# Autodesk Inventor assembly: BNT 2010-2.6 +1166L C7T-J1K_10000KBK 15BF 15
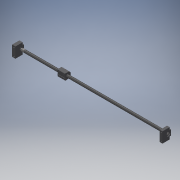
[picture p0: Inventor's stored thumbnail of the model, 180x180]
Saved by Autodesk Inventor 2018 (Build 220112000, 112)
## iProperties
Category: PARTsolutions
Company: THK
Created: 2017-05-30
Part Number: BNT 2010-2.6 +1166L C7T-J1K_10000KBK 15BF 15
Catalog Web Link: www.cadenas.de
Description: Rectangular-Nut Non-Preloaded Type BNT-
Vendor: THK
Document SubType Name: Assembly
Designer: psAdmin
Manufacturer: THK
Title: BNT 2010-2.6 +1166L C7T-J1K
Author: Cadenas PARTsolutions
## Documents named in this file (7)
- C:\Users\P300023\Documents\GitHub\CNC-Lathe-CAD2.0\CNC Lathe Project\Project Files\Updated Z axis\AIS2016\Z-AxisLong-Shaft-Final.iam
- C:\Users\P300023\Documents\GitHub\CNC-Lathe-CAD2.0\CNC Lathe Project\Project Files\Updated Z axis\AIS2016\BNT 2010-2_61000-J1K Shaft.ipt
- C:\Users\P300023\Documents\GitHub\CNC-Lathe-CAD2.0\CNC Lathe Project\Project Files\Updated Z axis\AIS2016\BNT 2010-2_6 Nut.ipt
- C:\Users\P300023\Documents\GitHub\CNC-Lathe-CAD2.0\CNC Lathe Project\Project Files\Updated Z axis\AIS2016\BK 15.ipt
- C:\Users\P300023\Documents\GitHub\CNC-Lathe-CAD2.0\CNC Lathe Project\Project Files\Updated Z axis\AIS2016\BK 15collar.ipt
- C:\Users\P300023\Documents\GitHub\CNC-Lathe-CAD2.0\CNC Lathe Project\Project Files\Updated Z axis\AIS2016\BF 15 Part2.ipt
- C:\Users\P300023\Documents\GitHub\CNC-Lathe-CAD2.0\CNC Lathe Project\Project Files\Updated Z axis\AIS2016\BF 15 Part1.ipt
## Components (6 placed, 6 different names)
1. BNT 2010-2_61000-J1K Shaft:1 — Mate:1
2. BNT 2010-2_6 Nut:1 — Mate:1
3. BK 15:1
4. BK 15collar:1
5. BF 15 Part2:1
6. BF 15 Part1:1
## Relationships (1: Mate 1)
- Mate:1: BNT 2010-2_61000-J1K Shaft:1 ↔ BNT 2010-2_6 Nut:1
